# Autodesk Inventor assembly: VelcroTrack2
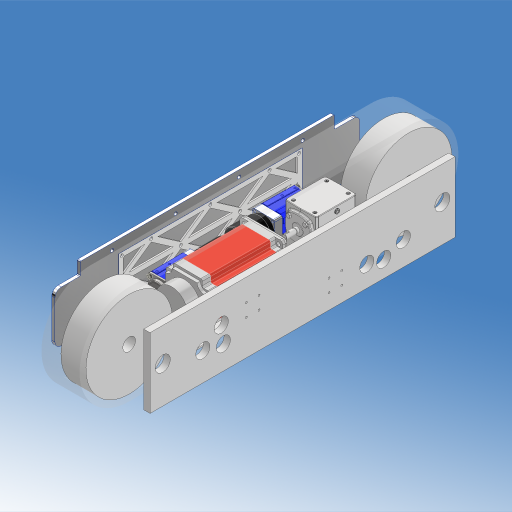
[picture p0: Inventor's stored thumbnail of the model, 512x512]
Saved by Autodesk Inventor 2024 (Build 280153000, 153)
## iProperties
Created: 2024-04-01
Part Number: VelcroTrack2
Document SubType Name: Assembly
Designer: seene
Author: seene
## Documents named in this file (10)
- C:\Users\seene\OneDrive\SBRT\Robocup Rescue\Drive\TestRigs\Other Ideas\VelcroTrack2.iam
- C:\Users\seene\OneDrive\SBRT\Robocup Rescue\Drive\v1\ChassisInterface.ipt
- C:\Users\seene\OneDrive\SBRT\Robocup Rescue\Drive\QuintinCAD\NEMA34_gearbox_sheetMetaMount - Copy.ipt
- C:\Users\seene\OneDrive\SBRT\Robocup Rescue\Drive\MasterSketch - Copy.ipt
- C:\Users\seene\OneDrive\SBRT\Robocup Rescue\Drive\TestRigs\MainDriveTestrig\MotorStandoff.ipt
- C:\Users\seene\OneDrive\SBRT\Robocup Rescue\Drive\v1\FlipperMotorGearboxAssembly.iam
- C:\Users\seene\OneDrive\SBRT\Robocup Rescue\Drive\TestRigs\MainDriveTestrig\Pulleys\BigPulley.ipt
- C:\Users\seene\OneDrive\SBRT\Robocup Rescue\Drive\MasterSketch - Copy - Copy.ipt
- C:\Users\seene\OneDrive\SBRT\Robocup Rescue\Drive\v1\QCI-34HC-3_v2.ipt
- C:\Users\seene\OneDrive\SBRT\Robocup Rescue\Drive\v1\5887K172_Right-Angle Speed Reducer.ipt
## Components (11 placed, 9 different names)
1. ChassisInterface:1 — Mate:1, Mate:2, Mate:9
2. NEMA34_gearbox_sheetMetaMount - Copy:1 — Mate:1, Mate:2, Mate:4, Mate:5, Mate:6, Mate:7, Mate:8, Mate:9, Flush:3, Mate:16, Mate:17, Mate:18
3. MasterSketch - Copy:1 — Mate:4, Mate:10, Mate:11, Flush:3
4. MotorStandoff:1 — Mate:5, Mate:6, Mate:14, Mate:15
5. FlipperMotorGearboxAssembly:1 [sub-assembly] — Mate:7
6. FlipperMotorGearboxAssembly:2 [sub-assembly] — Mate:8
7. BigPulley:1 — Mate:10, Flush:1, Mate:12
8. BigPulley:2 — Mate:11, Flush:1, Mate:13, Flush:2
9. MasterSketch - Copy - Copy:1 — Mate:12, Mate:13, Flush:2
10. QCI-34HC-3_v2:1 — Mate:14, Mate:15
11. 5887K172_Right-Angle Speed Reducer:1 — Mate:16, Mate:17, Mate:18
## Relationships (20: Mate 17, Flush 3)
- Mate:1: ChassisInterface:1 ↔ NEMA34_gearbox_sheetMetaMount - Copy:1
- Mate:2: ChassisInterface:1 ↔ NEMA34_gearbox_sheetMetaMount - Copy:1
- Mate:4 (19.05 mm): NEMA34_gearbox_sheetMetaMount - Copy:1 ↔ MasterSketch - Copy:1
- Mate:5: NEMA34_gearbox_sheetMetaMount - Copy:1 ↔ MotorStandoff:1
- Mate:6: NEMA34_gearbox_sheetMetaMount - Copy:1 ↔ MotorStandoff:1
- Mate:7: NEMA34_gearbox_sheetMetaMount - Copy:1 ↔ FlipperMotorGearboxAssembly:1
- Mate:8: NEMA34_gearbox_sheetMetaMount - Copy:1 ↔ FlipperMotorGearboxAssembly:2
- Mate:9: ChassisInterface:1 ↔ NEMA34_gearbox_sheetMetaMount - Copy:1
- Mate:10: MasterSketch - Copy:1 ↔ BigPulley:1
- Mate:11: MasterSketch - Copy:1 ↔ BigPulley:2
- Flush:1: BigPulley:1 ↔ BigPulley:2
- Mate:12: BigPulley:1 ↔ MasterSketch - Copy - Copy:1
- Mate:13: BigPulley:2 ↔ MasterSketch - Copy - Copy:1
- Flush:2: BigPulley:2 ↔ MasterSketch - Copy - Copy:1
- Flush:3 (-7.5366 mm): NEMA34_gearbox_sheetMetaMount - Copy:1 ↔ MasterSketch - Copy:1
- Mate:14: MotorStandoff:1 ↔ QCI-34HC-3_v2:1
- Mate:15: MotorStandoff:1 ↔ QCI-34HC-3_v2:1
- Mate:16: NEMA34_gearbox_sheetMetaMount - Copy:1 ↔ 5887K172_Right-Angle Speed Reducer:1
- Mate:17: NEMA34_gearbox_sheetMetaMount - Copy:1 ↔ 5887K172_Right-Angle Speed Reducer:1
- Mate:18: NEMA34_gearbox_sheetMetaMount - Copy:1 ↔ 5887K172_Right-Angle Speed Reducer:1
